# Autodesk Inventor assembly: BG005_huenin20_23
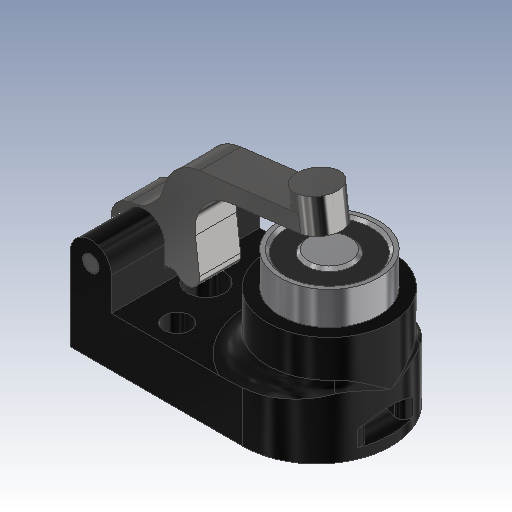
[picture p0: Inventor's stored thumbnail of the model, 512x512]
Saved by Autodesk Inventor 2023.3 (Build 273359000, 359)
## iProperties
Company: HTBLA Kaindorf
RuleStatus: InUse
Created: 2024-01-29
Part Number: BG005_huenin20_23
Project: Fiberprinter-Hotend
Material: Generisch
Description: SMN_Aktuator
Document SubType Name: Assembly
Designer: huenin20
Mass: 29.9088 g
Surface Area: 44.7984 cm^2
Volume: 5.54638 cm^3
Density: 5.39248 g/cm^3
AfterDocNew0: iProperties-Editor_aufrufen
Author: nicob
Keywords: 2023
## Documents named in this file (7)
- C:\Users\nicob\OneDrive\Dokumente\Kop\Fiberprinter_Hotend\BG005_huenin20_23_Fiberprinter-Hotend_SMN_Aktuator.iam
- C:\Users\nicob\OneDrive\Dokumente\Kop\Fiberprinter_Hotend\BT016_huenin20_23_Fiberprinter-Hotend_SMN_Aktuatorgehäuse.ipt
- C:\Users\nicob\OneDrive\Dokumente\Kop\Fiberprinter_Hotend\BT017_huenin20_23_Fiberprinter-Hotend_SMN_Aktuatorhebel.ipt
- C:\Users\nicob\OneDrive\Dokumente\Kop\Fiberprinter_Hotend\Elektromagnet.ipt
- C:\Users\nicob\OneDrive\Dokumente\Kop\Fiberprinter_Hotend\Normteile\de-DE\ISO 4762(2)\ISO 4762 - M3 x 5ISO.ipt
- C:\Users\nicob\OneDrive\Dokumente\Kop\Fiberprinter_Hotend\BT018_huenin20_23_Fiberprinter-Hotend_SMN_Aktuator_Führungshülse.ipt
- C:\Users\nicob\OneDrive\Dokumente\Kop\Fiberprinter_Hotend\Normteile\de-DE\ISO 2338(2)\ISO 2338 - 2 h8 x 18.ipt
## Components (6 placed, 6 different names)
1. BT016_huenin20_23_Fiberprinter-Hotend_SMN_Aktuatorgehäuse:1 — Einfügen:2, Einfügen:4, Einfügen:5, Einfügen:6, Einfügen:7
2. Elektromagnet:1 — Einfügen:2, Winkel:1
3. BT017_huenin20_23_Fiberprinter-Hotend_SMN_Aktuatorhebel:1 — Einfügen:5, Winkel:1
4. ISO 2338 2 h8 x 18:1 — Einfügen:4
5. ISO 4762 M3 x 5:1 — Einfügen:6
6. BT018_huenin20_23_Fiberprinter-Hotend_SMN_Aktuator_Führungshülse:1 — Einfügen:7
## Relationships (6: Insert 5, Angle 1)
- Einfügen:2 [Insert]: BT016_huenin20_23_Fiberprinter-Hotend_SMN_Aktuatorgehäuse:1 ↔ Elektromagnet:1
- Einfügen:4 [Insert]: BT016_huenin20_23_Fiberprinter-Hotend_SMN_Aktuatorgehäuse:1 ↔ ISO 2338 2 h8 x 18:1
- Einfügen:5 [Insert]: BT016_huenin20_23_Fiberprinter-Hotend_SMN_Aktuatorgehäuse:1 ↔ BT017_huenin20_23_Fiberprinter-Hotend_SMN_Aktuatorhebel:1
- Winkel:1 [Angle] (180 deg): Elektromagnet:1 ↔ BT017_huenin20_23_Fiberprinter-Hotend_SMN_Aktuatorhebel:1
- Einfügen:6 [Insert]: BT016_huenin20_23_Fiberprinter-Hotend_SMN_Aktuatorgehäuse:1 ↔ ISO 4762 M3 x 5:1
- Einfügen:7 [Insert]: BT016_huenin20_23_Fiberprinter-Hotend_SMN_Aktuatorgehäuse:1 ↔ BT018_huenin20_23_Fiberprinter-Hotend_SMN_Aktuator_Führungshülse:1
